# Autodesk Inventor assembly: 6in Colson Assem
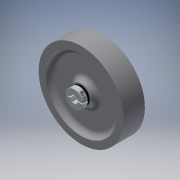
[picture p0: Inventor's stored thumbnail of the model, 180x180]
Saved by Autodesk Inventor 2019 (Build 230136000, 136)
## iProperties
Created: 2018-11-11
Part Number: 6in Colson Assem
Document SubType Name: Assembly
Designer: maste
Author: maste
## Documents named in this file (3)
- D:\Summer Drive Base V1\Summer Drivebase\6in Colson Assem.iam
- D:\Summer Drive Base V1\Summer Drivebase\colsonwgeelwithhub.iam
- D:\Summer Drive Base V1\Summer Drivebase\am-1238+Collar+Clamp,+0.5''+Hex+Bore,+Aluminum.iam
## Components (2 placed, 2 different names)
1. colsonwgeelwithhub:1 [sub-assembly] — Mate:1, Flush:1, Flush:2
2. am-1238+Collar+Clamp,+0.5''+Hex+Bore,+Aluminum:1 [sub-assembly] — Mate:1, Flush:1, Flush:2
## Relationships (3: Flush 2, Mate 1)
- Mate:1: colsonwgeelwithhub:1 ↔ am-1238+Collar+Clamp,+0.5''+Hex+Bore,+Aluminum:1
- Flush:1: colsonwgeelwithhub:1 ↔ am-1238+Collar+Clamp,+0.5''+Hex+Bore,+Aluminum:1
- Flush:2: colsonwgeelwithhub:1 ↔ am-1238+Collar+Clamp,+0.5''+Hex+Bore,+Aluminum:1
